# Autodesk Inventor assembly: Placa USB-B
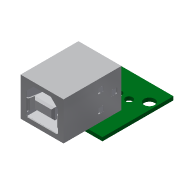
[picture p0: Inventor's stored thumbnail of the model, 180x180]
Saved by Autodesk Inventor 2020 (Build 240168000, 168)
## iProperties
Created: 2012-05-07
Part Number: Placa USB-B
Document SubType Name: Assembly
Designer: sdarley
Author: sdarley
## Documents named in this file (5)
- C:\Users\Usuario\Desktop\Ensamble Ajust Fino Total + Elect. - Act. 19_10_2020 - copia\Componentes Electrónicos\Placa USB-B.iam
- C:\Users\Usuario\Desktop\Ensamble Ajust Fino Total + Elect. - Act. 19_10_2020 - copia\Componentes Electrónicos\USB Series B Receptacle Metal Shell.ipt
- C:\Users\Usuario\Desktop\Ensamble Ajust Fino Total + Elect. - Act. 19_10_2020 - copia\Componentes Electrónicos\USB Series B Receptacle Housing.ipt
- C:\Users\Usuario\Desktop\Ensamble Ajust Fino Total + Elect. - Act. 19_10_2020 - copia\Componentes Electrónicos\USB Series B Receptacle Terminal.ipt
- C:\Users\Usuario\Desktop\Ensamble Ajust Fino Total + Elect. - Act. 19_10_2020 - copia\Componentes Electrónicos\PCB USB-B Hembra.ipt
## Components (7 placed, 4 different names)
1. USB Series B Receptacle Metal Shell:1 — Mate:1, Mate:2, Flush:1, Flush:2, Mate:3, Mate:4, Mate:5, Mate:18, Flush:4, Flush:5
2. USB Series B Receptacle Housing:1 — Flush:2, Mate:3, Mate:4, Mate:5, Flush:3, Mate:6, Mate:7, Mate:8, Mate:9, Mate:10, Mate:11, Mate:12, Mate:13, Mate:14, Mate:15, Mate:16, Mate:17
3. USB Series B Receptacle Terminal:1 — Flush:3, Mate:6, Mate:7, Mate:8
4. USB Series B Receptacle Terminal:2 — Mate:9, Mate:16, Mate:17
5. USB Series B Receptacle Terminal:3 — Mate:10, Mate:12, Mate:13
6. USB Series B Receptacle Terminal:4 — Mate:11, Mate:14, Mate:15
7. PCB USB-B Hembra:1 — Mate:18, Flush:4, Flush:5
## Relationships (23: Mate 18, Flush 5)
- Mate:1: USB Series B Receptacle Metal Shell:1
- Mate:2: USB Series B Receptacle Metal Shell:1
- Flush:1: USB Series B Receptacle Metal Shell:1
- Flush:2: USB Series B Receptacle Metal Shell:1 ↔ USB Series B Receptacle Housing:1
- Mate:3: USB Series B Receptacle Metal Shell:1 ↔ USB Series B Receptacle Housing:1
- Mate:4: USB Series B Receptacle Metal Shell:1 ↔ USB Series B Receptacle Housing:1
- Mate:5: USB Series B Receptacle Metal Shell:1 ↔ USB Series B Receptacle Housing:1
- Flush:3: USB Series B Receptacle Housing:1 ↔ USB Series B Receptacle Terminal:1
- Mate:6: USB Series B Receptacle Housing:1 ↔ USB Series B Receptacle Terminal:1
- Mate:7: USB Series B Receptacle Housing:1 ↔ USB Series B Receptacle Terminal:1
- Mate:8: USB Series B Receptacle Housing:1 ↔ USB Series B Receptacle Terminal:1
- Mate:9: USB Series B Receptacle Housing:1 ↔ USB Series B Receptacle Terminal:2
- Mate:10: USB Series B Receptacle Housing:1 ↔ USB Series B Receptacle Terminal:3
- Mate:11: USB Series B Receptacle Housing:1 ↔ USB Series B Receptacle Terminal:4
- Mate:12: USB Series B Receptacle Housing:1 ↔ USB Series B Receptacle Terminal:3
- Mate:13: USB Series B Receptacle Housing:1 ↔ USB Series B Receptacle Terminal:3
- Mate:14: USB Series B Receptacle Housing:1 ↔ USB Series B Receptacle Terminal:4
- Mate:15: USB Series B Receptacle Housing:1 ↔ USB Series B Receptacle Terminal:4
- Mate:16: USB Series B Receptacle Housing:1 ↔ USB Series B Receptacle Terminal:2
- Mate:17: USB Series B Receptacle Housing:1 ↔ USB Series B Receptacle Terminal:2
- Mate:18: USB Series B Receptacle Metal Shell:1 ↔ PCB USB-B Hembra:1
- Flush:4 (3.95 mm): USB Series B Receptacle Metal Shell:1 ↔ PCB USB-B Hembra:1
- Flush:5 (10.7 mm): USB Series B Receptacle Metal Shell:1 ↔ PCB USB-B Hembra:1
